# Autodesk Inventor assembly: 000.100 - Сборка ходовой рамы
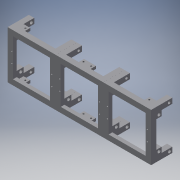
[picture p0: Inventor's stored thumbnail of the model, 180x180]
Saved by Autodesk Inventor 2019 (Build 230136000, 136)
## iProperties
Created: 2020-06-05
Part Number: 000.100 - Сборка ходовой рамы
Material: Типовые
Document SubType Name: Assembly
Designer: Петров Иван
Author: Петров Иван
## Documents named in this file (3)
- E:\IVAN\Ivan_desktop\My_projects\RTK\000.100 - Сборка ходовой рамы.iam
- E:\IVAN\Ivan_desktop\My_projects\RTK\000.102 - Центральный сегмент ходовой части.ipt
- E:\IVAN\Ivan_desktop\My_projects\RTK\000.101 - Крайний сегмент ходовой части.ipt
## Components (3 placed, 2 different names)
1. 000.102 - Центральный сегмент ходовой части:1 — Совмещение:1, Заподлицо:1, Совмещение:2, Совмещение:3, Совмещение:4, Совмещение:5, Совмещение:6, Совмещение:7, Совмещение:8
2. 000.101 - Крайний сегмент ходовой части:1 — Совмещение:5, Совмещение:6, Совмещение:7
3. 000.101 - Крайний сегмент ходовой части:2 — Совмещение:2, Совмещение:3, Совмещение:4
## Relationships (9: Mate 8, Flush 1)
- Совмещение:1 [Mate] (-45 mm): 000.102 - Центральный сегмент ходовой части:1
- Заподлицо:1 [Flush] (-45 mm): 000.102 - Центральный сегмент ходовой части:1
- Совмещение:2 [Mate]: 000.102 - Центральный сегмент ходовой части:1 ↔ 000.101 - Крайний сегмент ходовой части:2
- Совмещение:3 [Mate]: 000.102 - Центральный сегмент ходовой части:1 ↔ 000.101 - Крайний сегмент ходовой части:2
- Совмещение:4 [Mate]: 000.102 - Центральный сегмент ходовой части:1 ↔ 000.101 - Крайний сегмент ходовой части:2
- Совмещение:5 [Mate]: 000.102 - Центральный сегмент ходовой части:1 ↔ 000.101 - Крайний сегмент ходовой части:1
- Совмещение:6 [Mate]: 000.102 - Центральный сегмент ходовой части:1 ↔ 000.101 - Крайний сегмент ходовой части:1
- Совмещение:7 [Mate]: 000.102 - Центральный сегмент ходовой части:1 ↔ 000.101 - Крайний сегмент ходовой части:1
- Совмещение:8 [Mate]: 000.102 - Центральный сегмент ходовой части:1
